# Autodesk Inventor assembly: Kinematic-Mount Back
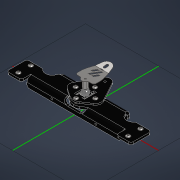
[picture p0: Inventor's stored thumbnail of the model, 180x180]
Saved by Autodesk Inventor 2022.2 (Build 262287010, 287A)
## iProperties
Created: 2022-03-13
Part Number: Kinematic-Mount Back
Document SubType Name: Assembly
Designer: sleib
Author: sleib
## Documents named in this file (8)
- C:\Users\sleib\Projekte\Voron-2\CAD\Inventor\Kinematic-Mount Back.iam
- C:\Users\sleib\Projekte\Voron-2\CAD\Inventor\Kinematic-Bed Back-Support Bottom.ipt
- C:\Users\sleib\Projekte\Voron-2\CAD\Inventor\Pin 5x15.ipt
- C:\Users\sleib\Projekte\Voron-2\CAD\Inventor\Kinematic-Bed Back-Support Top.ipt
- C:\Users\sleib\Projekte\Voron-2\CAD\Inventor\M3x8 BHCS.ipt
- C:\Users\sleib\Projekte\Voron-2\CAD\Inventor\M3 Threaded Ball.ipt
- C:\Users\sleib\Projekte\Voron-2\CAD\Inventor\M3x10x6 Standoff.ipt
- C:\Users\sleib\Projekte\Voron-2\CAD\Inventor\Kinematic-Bed Leaf-Spring.ipt
## Components (15 placed, 7 different names)
1. Kinematic-Bed Back-Support Bottom:1 — Passend:1, Passend:3, Passend:4, Passend:5, Passend:6, Passend:7, Passend:8, Passend:9, Passend:10, Passend:11, Passend:12, Passend:20, Passend:21, Passend:22, Passend:23, Passend:36, Passend:37, Passend:38, Passend:39, Passend:40, Passend:41, Passend:42, Passend:43
2. Kinematic-Bed Back-Support Top:1 — Passend:13, Passend:14, Passend:15, Passend:16, Passend:17, Passend:19, Passend:24, Passend:25, Passend:26, Passend:27, Passend:28, Passend:35
3. M3 Threaded Ball:1 — Tangential:1, Tangential:2, Passend:29, Passend:30
4. M3x10x6 Standoff:1 — Passend:29, Passend:30, Passend:31, Passend:32
5. Kinematic-Bed Leaf-Spring:1 — Passend:31, Passend:32, Passend:35
6. Pin 5x15:1 — Passend:9, Passend:10, Passend:11, Passend:14, Tangential:2
7. Pin 5x15:2 — Passend:7, Passend:8, Passend:12, Passend:13, Passend:15, Tangential:1
8. M3x8 BHCS:1 — Passend:19, Passend:21, Passend:26
9. M3x8 BHCS:2 — Passend:20, Passend:27, Passend:28
10. M3x8 BHCS:3 — Passend:17, Passend:23, Passend:25
11. M3x8 BHCS:4 — Passend:16, Passend:22, Passend:24
12. M3x8 BHCS:5 — Passend:36, Passend:40
13. M3x8 BHCS:6 — Passend:37, Passend:41
14. M3x8 BHCS:7 — Passend:38, Passend:42
15. M3x8 BHCS:8 — Passend:39, Passend:43
## Relationships (41: Mate 39, Tangent 2)
- Passend:1 [Mate]: Kinematic-Bed Back-Support Bottom:1
- Passend:3 [Mate]: Kinematic-Bed Back-Support Bottom:1
- Passend:4 [Mate]: Kinematic-Bed Back-Support Bottom:1
- Passend:5 [Mate]: Kinematic-Bed Back-Support Bottom:1
- Passend:6 [Mate]: Kinematic-Bed Back-Support Bottom:1
- Passend:7 [Mate] (2.5 mm): Kinematic-Bed Back-Support Bottom:1 ↔ Pin 5x15:2
- Passend:8 [Mate] (2.5 mm): Kinematic-Bed Back-Support Bottom:1 ↔ Pin 5x15:2
- Passend:9 [Mate] (2.5 mm): Kinematic-Bed Back-Support Bottom:1 ↔ Pin 5x15:1
- Passend:10 [Mate] (2.5 mm): Kinematic-Bed Back-Support Bottom:1 ↔ Pin 5x15:1
- Passend:11 [Mate] (0.2 mm): Kinematic-Bed Back-Support Bottom:1 ↔ Pin 5x15:1
- Passend:12 [Mate] (0.2 mm): Kinematic-Bed Back-Support Bottom:1 ↔ Pin 5x15:2
- Passend:13 [Mate] (2.5 mm): Kinematic-Bed Back-Support Top:1 ↔ Pin 5x15:2
- Passend:14 [Mate] (2.5 mm): Kinematic-Bed Back-Support Top:1 ↔ Pin 5x15:1
- Passend:15 [Mate] (0.2 mm): Kinematic-Bed Back-Support Top:1 ↔ Pin 5x15:2
- Passend:16 [Mate]: Kinematic-Bed Back-Support Top:1 ↔ M3x8 BHCS:4
- Passend:17 [Mate]: Kinematic-Bed Back-Support Top:1 ↔ M3x8 BHCS:3
- Passend:19 [Mate]: Kinematic-Bed Back-Support Top:1 ↔ M3x8 BHCS:1
- Passend:20 [Mate]: Kinematic-Bed Back-Support Bottom:1 ↔ M3x8 BHCS:2
- Passend:21 [Mate]: Kinematic-Bed Back-Support Bottom:1 ↔ M3x8 BHCS:1
- Passend:22 [Mate]: Kinematic-Bed Back-Support Bottom:1 ↔ M3x8 BHCS:4
- Passend:23 [Mate]: Kinematic-Bed Back-Support Bottom:1 ↔ M3x8 BHCS:3
- Passend:24 [Mate]: Kinematic-Bed Back-Support Top:1 ↔ M3x8 BHCS:4
- Passend:25 [Mate]: Kinematic-Bed Back-Support Top:1 ↔ M3x8 BHCS:3
- Passend:26 [Mate]: Kinematic-Bed Back-Support Top:1 ↔ M3x8 BHCS:1
- Passend:27 [Mate]: Kinematic-Bed Back-Support Top:1 ↔ M3x8 BHCS:2
- Passend:28 [Mate]: Kinematic-Bed Back-Support Top:1 ↔ M3x8 BHCS:2
- Tangential:1: M3 Threaded Ball:1 ↔ Pin 5x15:2
- Tangential:2: M3 Threaded Ball:1 ↔ Pin 5x15:1
- Passend:29 [Mate]: M3 Threaded Ball:1 ↔ M3x10x6 Standoff:1
- Passend:30 [Mate] (1 mm): M3 Threaded Ball:1 ↔ M3x10x6 Standoff:1
- Passend:31 [Mate]: M3x10x6 Standoff:1 ↔ Kinematic-Bed Leaf-Spring:1
- Passend:32 [Mate]: M3x10x6 Standoff:1 ↔ Kinematic-Bed Leaf-Spring:1
- Passend:35 [Mate]: Kinematic-Bed Back-Support Top:1 ↔ Kinematic-Bed Leaf-Spring:1
- Passend:36 [Mate]: Kinematic-Bed Back-Support Bottom:1 ↔ M3x8 BHCS:5
- Passend:37 [Mate]: Kinematic-Bed Back-Support Bottom:1 ↔ M3x8 BHCS:6
- Passend:38 [Mate]: Kinematic-Bed Back-Support Bottom:1 ↔ M3x8 BHCS:7
- Passend:39 [Mate]: Kinematic-Bed Back-Support Bottom:1 ↔ M3x8 BHCS:8
- Passend:40 [Mate]: Kinematic-Bed Back-Support Bottom:1 ↔ M3x8 BHCS:5
- Passend:41 [Mate]: Kinematic-Bed Back-Support Bottom:1 ↔ M3x8 BHCS:6
- Passend:42 [Mate]: Kinematic-Bed Back-Support Bottom:1 ↔ M3x8 BHCS:7
- Passend:43 [Mate]: Kinematic-Bed Back-Support Bottom:1 ↔ M3x8 BHCS:8
